# Autodesk Inventor assembly: ASY PNS-002 right module
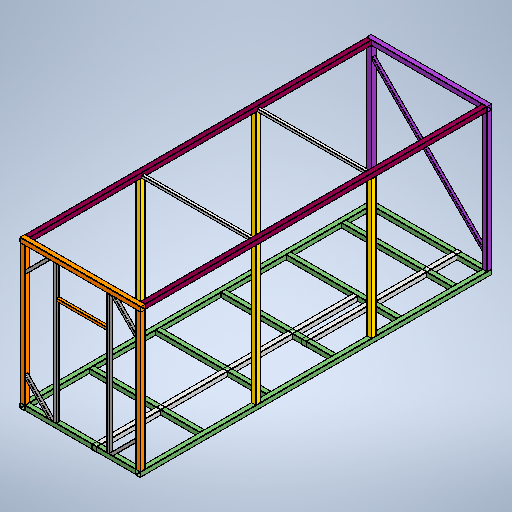
[picture p0: Inventor's stored thumbnail of the model, 512x512]
Saved by Autodesk Inventor 2025 (Build 290162010, 162A)
## iProperties
Created: 2025-03-25
Part Number: ASY PNS-002 right module
Document SubType Name: Assembly
Designer: user
Author: user
## Documents named in this file (7)
- C:\Users\admin\YandexDisk-badmisterfox\home pc\Inventor\PNS-Panaevsk\ASY PNS-002 right module.iam
- C:\Users\admin\YandexDisk-badmisterfox\home pc\Inventor\PNS-Panaevsk\ASY PNS-0210 frame right floor.iam
- C:\Users\admin\YandexDisk-badmisterfox\home pc\Inventor\PNS-Panaevsk\ASY PNS-0250 frame featheredge.iam
- C:\Users\admin\YandexDisk-badmisterfox\home pc\Inventor\PNS-Panaevsk\ASY PNS-0250 frame featheredge 0270.iam
- C:\Users\admin\YandexDisk-badmisterfox\home pc\Inventor\PNS-Panaevsk\PNS-0261 Upper beam.ipt
- C:\Users\admin\YandexDisk-badmisterfox\home pc\Inventor\PNS-Panaevsk\PNS-0262 middle pillar.ipt
- C:\Users\admin\YandexDisk-badmisterfox\home pc\Inventor\PNS-Panaevsk\PNS-0262 cross beam.ipt
## Components (11 placed, 6 different names)
1. ASY PNS-0210 frame right floor:1 [sub-assembly] — Rigid:3
2. ASY PNS-0250 frame featheredge:1 [sub-assembly] — Rigid:4, Rigid:5, Rigid:6, Rigid:7
3. ASY PNS-0250 frame featheredge 0270:1 [sub-assembly] — Rigid:3, Rigid:8, Rigid:9
4. PNS-0261 Upper beam:1 — Rigid:4
5. PNS-0261 Upper beam:2 — Rigid:5
6. PNS-0262 middle pillar:1 — Rigid:6
7. PNS-0262 middle pillar:2 — Rigid:7, Rigid:10
8. PNS-0262 middle pillar:3 — Rigid:8
9. PNS-0262 middle pillar:4 — Rigid:9, Rigid:11
10. PNS-0262 cross beam:1 — Rigid:11
11. PNS-0262 cross beam:2 — Rigid:10
## Relationships (10: WeldJoint 10)
- [WeldJoint]: ASY PNS-0210 frame right floor:1 ↔ ASY PNS-0250 frame featheredge:1
- Rigid:3 [WeldJoint]: ASY PNS-0210 frame right floor:1 ↔ ASY PNS-0250 frame featheredge 0270:1
- Rigid:4 [WeldJoint]: ASY PNS-0250 frame featheredge:1 ↔ PNS-0261 Upper beam:1
- Rigid:5 [WeldJoint]: ASY PNS-0250 frame featheredge:1 ↔ PNS-0261 Upper beam:2
- Rigid:6 [WeldJoint] (2200 mm): ASY PNS-0250 frame featheredge:1 ↔ PNS-0262 middle pillar:1
- Rigid:7 [WeldJoint] (2200 mm): ASY PNS-0250 frame featheredge:1 ↔ PNS-0262 middle pillar:2
- Rigid:8 [WeldJoint] (2200 mm): ASY PNS-0250 frame featheredge 0270:1 ↔ PNS-0262 middle pillar:3
- Rigid:9 [WeldJoint] (2200 mm): ASY PNS-0250 frame featheredge 0270:1 ↔ PNS-0262 middle pillar:4
- Rigid:10 [WeldJoint]: PNS-0262 middle pillar:2 ↔ PNS-0262 cross beam:2
- Rigid:11 [WeldJoint]: PNS-0262 middle pillar:4 ↔ PNS-0262 cross beam:1
